# Autodesk Inventor assembly: EDM Middle Shield
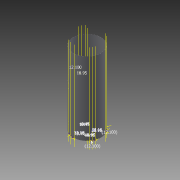
[picture p0: Inventor's stored thumbnail of the model, 180x180]
Saved by Autodesk Inventor 2015 (Build 190159000, 159)
## iProperties
Created: 2014-06-19
Part Number: EDM Middle Shield
Document SubType Name: Assembly
Designer: Aki
Author: Aki
## Documents named in this file (5)
- C:\ColdMatter\CADFiles\EDM Machine\EDM Middle Shield\EDM Middle Shield.iam
- C:\ColdMatter\CADFiles\EDM Machine\EDM Middle Shield\EDM Middle Shield Part 1.ipt
- C:\ColdMatter\CADFiles\EDM Machine\EDM Middle Shield\EDM Middle Shield Part 2.ipt
- C:\ColdMatter\CADFiles\EDM Machine\EDM Middle Shield\EDM Middle Shield Part 3.ipt
- C:\ColdMatter\CADFiles\EDM Machine\EDM Middle Shield\EDM Middle Shield Part 4.ipt
## Components (4 placed, 4 different names)
1. EDM Middle Shield Part 3:1 — Mate:10, Mate:12, Mate:13
2. EDM Middle Shield Part 4:1 — Mate:10, Mate:11, Mate:14
3. EDM Middle Shield Part 2:1 — Mate:11, Mate:12, Mate:13, Mate:15, Mate:16
4. EDM Middle Shield Part 1:1 — Mate:14, Mate:15, Mate:16
## Relationships (7: Mate 7)
- Mate:10: EDM Middle Shield Part 3:1 ↔ EDM Middle Shield Part 4:1
- Mate:11: EDM Middle Shield Part 4:1 ↔ EDM Middle Shield Part 2:1
- Mate:12: EDM Middle Shield Part 3:1 ↔ EDM Middle Shield Part 2:1
- Mate:13: EDM Middle Shield Part 3:1 ↔ EDM Middle Shield Part 2:1
- Mate:14: EDM Middle Shield Part 4:1 ↔ EDM Middle Shield Part 1:1
- Mate:15: EDM Middle Shield Part 2:1 ↔ EDM Middle Shield Part 1:1
- Mate:16: EDM Middle Shield Part 2:1 ↔ EDM Middle Shield Part 1:1
